# Autodesk Inventor assembly: Gear Set WIthout Spacer
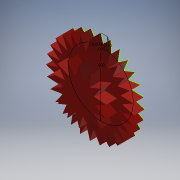
[picture p0: Inventor's stored thumbnail of the model, 180x180]
Saved by Autodesk Inventor 2018.3 (Build 223284000, 284)
## iProperties
Created: 2018-09-18
Part Number: Gear Set WIthout Spacer
Document SubType Name: Assembly
Designer: User
Author: User
## Documents named in this file (3)
- D:\Gear Set WIthout Spacer.iam
- D:\Big Gear Phone Case Mech.ipt
- D:\Small Gear Phone Case Mech.ipt
## Components (2 placed, 2 different names)
1. Big Gear Phone Case Mech:1 — Insert:1
2. Small Gear Phone Case Mech:1 — Insert:1
## Relationships (1: Insert 1)
- Insert:1: Big Gear Phone Case Mech:1 ↔ Small Gear Phone Case Mech:1
